# Autodesk Inventor assembly: Ensamblaje extra
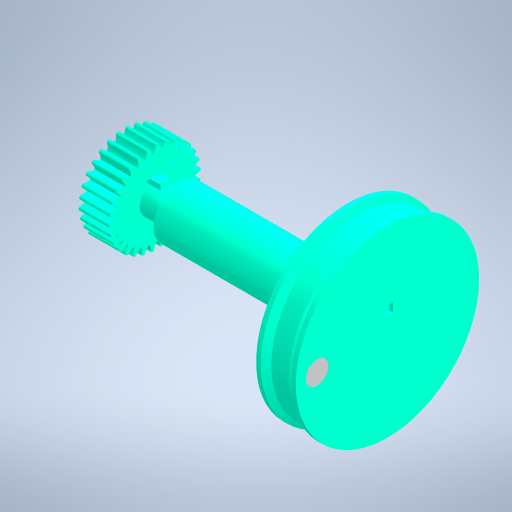
[picture p0: Inventor's stored thumbnail of the model, 512x512]
Saved by Autodesk Inventor 2024 (Build 280153000, 153)
## iProperties
Created: 2024-03-25
Part Number: Ensamblaje extra
Document SubType Name: Assembly
Designer: Alexa
Author: Alexa
## Documents named in this file (6)
- C:\Users\Alexa\OneDrive\Documentos\Universidad 2024\Dinámica\Lab dinámica\Ensamblaje extra.iam
- C:\Users\Alexa\Downloads\EJE_CUÑEROS.ipt
- C:\Users\Alexa\Downloads\ENGRANE.ipt
- C:\Users\Alexa\Downloads\POLEA.ipt
- C:\Users\Alexa\Downloads\CUÑA.ipt
- C:\Users\Alexa\OneDrive\Documentos\Universidad 2024\Dinámica\Lab dinámica\pieza extra ensamble v2.ipt
## Components (6 placed, 5 different names)
1. EJE_CUÑEROS:1 — Insertar:1, Insertar:2, Coincidencia:1, Coincidencia:2, Coincidencia:3, Coincidencia:4, Rígido:1, Plana:1
2. ENGRANE:1 — Insertar:2, Coincidencia:3, Coincidencia:4
3. POLEA:1 — Insertar:1, Coincidencia:1, Coincidencia:2, Coincidencia:5
4. CUÑA:2 — Rígido:1
5. CUÑA:3 — Plana:1
6. pieza extra ensamble v2:1 — Coincidencia:5
## Relationships (9: Mate 5, Insert 2, WeldJoint 1, PlanarJoint 1)
- Insertar:1: EJE_CUÑEROS:1 ↔ POLEA:1
- Insertar:2: EJE_CUÑEROS:1 ↔ ENGRANE:1
- Coincidencia:1 [Mate]: EJE_CUÑEROS:1 ↔ POLEA:1
- Coincidencia:2 [Mate]: EJE_CUÑEROS:1 ↔ POLEA:1
- Coincidencia:3 [Mate]: EJE_CUÑEROS:1 ↔ ENGRANE:1
- Coincidencia:4 [Mate]: EJE_CUÑEROS:1 ↔ ENGRANE:1
- Rígido:1 [WeldJoint]: EJE_CUÑEROS:1 ↔ CUÑA:2
- Plana:1: EJE_CUÑEROS:1 ↔ CUÑA:3
- Coincidencia:5 [Mate]: POLEA:1 ↔ pieza extra ensamble v2:1
